# Autodesk Inventor assembly: Raspberry Pi 4B with heatsink
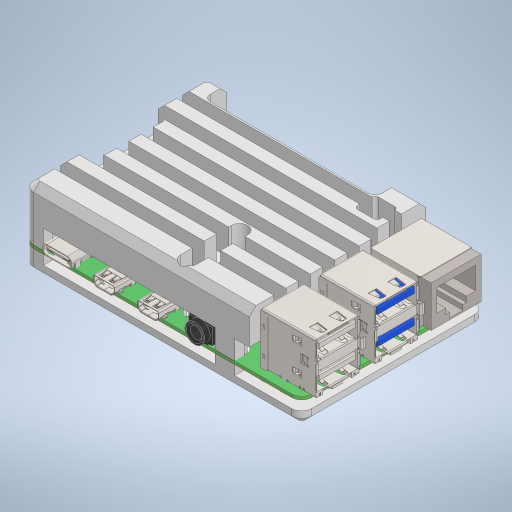
[picture p0: Inventor's stored thumbnail of the model, 512x512]
Saved by Autodesk Inventor 2023 (Build 270158000, 158)
## iProperties
Created: 2023-04-11
Part Number: Raspberry Pi 4B with heatsink
Document SubType Name: Assembly
Designer: ASARe-DAQ-PC
Author: ASARe-DAQ-PC
## Documents named in this file (4)
- D:\EB camera\model of EB camera\for manufacture\Raspberry Pi 4B with heatsink.iam
- D:\EB camera\model of EB camera\for manufacture\User Library-Raspberry-Pi-4-Model-B-03.ipt
- D:\EB camera\model of EB camera\for manufacture\Raspberry-Pi-4B heatsink1.ipt
- D:\EB camera\model of EB camera\for manufacture\Raspberry-Pi-4B heatsink2.ipt
## Components (3 placed, 3 different names)
1. User Library-Raspberry-Pi-4-Model-B-03:1 — Insert:1, Insert:2, Insert:3, Insert:4, Insert:5, Insert:6
2. Raspberry-Pi-4B heatsink1:1 — Insert:1, Insert:2, Insert:3, Insert:4
3. Raspberry-Pi-4B heatsink2:1 — Insert:5, Insert:6
## Relationships (6: Insert 6)
- Insert:1: User Library-Raspberry-Pi-4-Model-B-03:1 ↔ Raspberry-Pi-4B heatsink1:1
- Insert:2: User Library-Raspberry-Pi-4-Model-B-03:1 ↔ Raspberry-Pi-4B heatsink1:1
- Insert:3: User Library-Raspberry-Pi-4-Model-B-03:1 ↔ Raspberry-Pi-4B heatsink1:1
- Insert:4: User Library-Raspberry-Pi-4-Model-B-03:1 ↔ Raspberry-Pi-4B heatsink1:1
- Insert:5: User Library-Raspberry-Pi-4-Model-B-03:1 ↔ Raspberry-Pi-4B heatsink2:1
- Insert:6: User Library-Raspberry-Pi-4-Model-B-03:1 ↔ Raspberry-Pi-4B heatsink2:1
